# Autodesk Inventor assembly: slider for Reflection
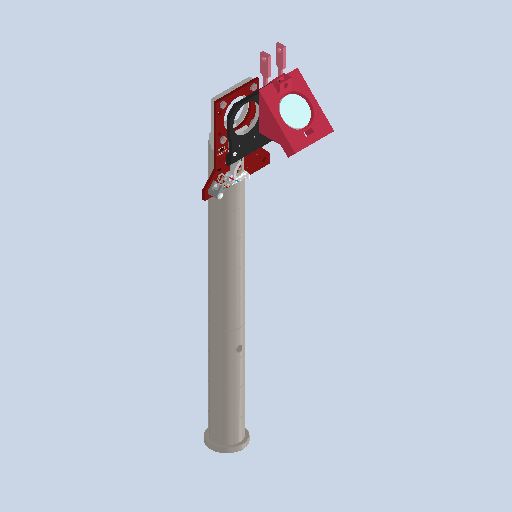
[picture p0: Inventor's stored thumbnail of the model, 512x512]
Saved by Autodesk Inventor 2026.1 (Build 301233000, 233)
## iProperties
Created: 2025-06-02
Part Number: slider for Reflection
Document SubType Name: Assembly
Designer: Julian
Author: Julian
## Documents named in this file (9)
- C:\Users\user\Desktop\setup for publishing\slider for Reflection.iam
- C:\Users\user\Desktop\setup for publishing\ELL6.ipt
- C:\Users\user\Desktop\setup for publishing\Newport-M-PS-4-1.ipt
- C:\Users\user\Desktop\setup for publishing\Newport-M-PS-6E-.ipt
- C:\Users\user\Desktop\setup for publishing\RS4_M.ipt
- C:\Users\user\Desktop\setup for publishing\ELLA1-Step.ipt
- C:\Users\user\Desktop\setup for publishing\SpiegelSlider.ipt
- C:\Users\user\Desktop\setup for publishing\Klemme für SpiegelSlider.ipt
- C:\Users\user\Desktop\setup for publishing\BB1-E02.ipt
## Components (8 placed, 8 different names)
1. ELL6:1 — Passend:1, Passend:2, Passend:3, Passend:13, Passend:14, Passend:15
2. Newport-M-PS-4-1:1 — Passend:4, Passend:5
3. Newport-M-PS-6E-:1 — Passend:4, Passend:5, Passend:6, Passend:7
4. RS4_M:1 — Passend:6, Passend:7, Passend:8, Passend:9
5. ELLA1-Step:1 — Passend:1, Passend:2, Passend:3, Passend:8, Passend:9
6. SpiegelSlider:1 — Passend:10, Passend:11, Passend:12, Passend:13, Passend:14
7. Klemme für SpiegelSlider:1 — Passend:12, Passend:15
8. BB1-E02:1 — Passend:10, Passend:11
## Relationships (15: Mate 15)
- Passend:1 [Mate]: ELL6:1 ↔ ELLA1-Step:1
- Passend:2 [Mate]: ELL6:1 ↔ ELLA1-Step:1
- Passend:3 [Mate]: ELL6:1 ↔ ELLA1-Step:1
- Passend:4 [Mate]: Newport-M-PS-4-1:1 ↔ Newport-M-PS-6E-:1
- Passend:5 [Mate]: Newport-M-PS-4-1:1 ↔ Newport-M-PS-6E-:1
- Passend:6 [Mate]: Newport-M-PS-6E-:1 ↔ RS4_M:1
- Passend:7 [Mate]: Newport-M-PS-6E-:1 ↔ RS4_M:1
- Passend:8 [Mate]: RS4_M:1 ↔ ELLA1-Step:1
- Passend:9 [Mate]: RS4_M:1 ↔ ELLA1-Step:1
- Passend:10 [Mate]: SpiegelSlider:1 ↔ BB1-E02:1
- Passend:11 [Mate]: SpiegelSlider:1 ↔ BB1-E02:1
- Passend:12 [Mate]: SpiegelSlider:1 ↔ Klemme für SpiegelSlider:1
- Passend:13 [Mate]: ELL6:1 ↔ SpiegelSlider:1
- Passend:14 [Mate]: ELL6:1 ↔ SpiegelSlider:1
- Passend:15 [Mate]: ELL6:1 ↔ Klemme für SpiegelSlider:1
